# Autodesk Inventor assembly: Mass 2, 3 Group
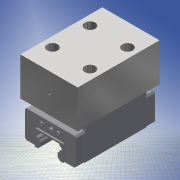
[picture p0: Inventor's stored thumbnail of the model, 180x180]
Saved by Autodesk Inventor 2016 (Build 200138000, 138)
## iProperties
Created: 2015-07-07
Part Number: Mass 2, 3 Group
Document SubType Name: Assembly
Designer: Dennis
Mass: 4113.68 g
Surface Area: 687.354 cm^2
Volume: 527.98 cm^3
Density: 7.79135 g/cm^3
Author: Dennis
## Documents named in this file (4)
- C:\Users\Jason\Dropbox\NI Work\NI Ball Bearing Slider Crank\CAD\Assemblies\Mass 2, 3 Group.iam
- C:\Users\Jason\Dropbox\NI Work\NI Ball Bearing Slider Crank\CAD\Mass 2, 3.ipt
- C:\Users\Jason\Dropbox\NI Work\NI Ball Bearing Slider Crank\CAD\McMaster Parts\Ball Bearing Carriage - Ball-Bearing Carriage, Threaded-Hole, for 34 mm Rail Width - 6709K21.ipt
- C:\Users\Jason\Dropbox\NI Work\NI Ball Bearing Slider Crank\CAD\McMaster Parts\M8x1.25x50.ipt
## Components (6 placed, 3 different names)
1. Mass 2, 3:1 — Mate:1, Mate:2, Mate:3, Mate:4, Mate:5, Mate:6, Mate:7, Mate:8, Mate:9, Mate:10, Mate:11
2. Ball Bearing Carriage - Ball-Bearing Carriage, Threaded-Hole, for 34 mm Rail Width - 6709K21:1 — Mate:1, Mate:2, Mate:3
3. M8x1.25x50:1 — Mate:4, Mate:8
4. M8x1.25x50:2 — Mate:5, Mate:9
5. M8x1.25x50:3 — Mate:6, Mate:10
6. M8x1.25x50:4 — Mate:7, Mate:11
## Relationships (11: Mate 11)
- Mate:1: Mass 2, 3:1 ↔ Ball Bearing Carriage - Ball-Bearing Carriage, Threaded-Hole, for 34 mm Rail Width - 6709K21:1
- Mate:2: Mass 2, 3:1 ↔ Ball Bearing Carriage - Ball-Bearing Carriage, Threaded-Hole, for 34 mm Rail Width - 6709K21:1
- Mate:3: Mass 2, 3:1 ↔ Ball Bearing Carriage - Ball-Bearing Carriage, Threaded-Hole, for 34 mm Rail Width - 6709K21:1
- Mate:4: Mass 2, 3:1 ↔ M8x1.25x50:1
- Mate:5: Mass 2, 3:1 ↔ M8x1.25x50:2
- Mate:6: Mass 2, 3:1 ↔ M8x1.25x50:3
- Mate:7: Mass 2, 3:1 ↔ M8x1.25x50:4
- Mate:8: Mass 2, 3:1 ↔ M8x1.25x50:1
- Mate:9: Mass 2, 3:1 ↔ M8x1.25x50:2
- Mate:10: Mass 2, 3:1 ↔ M8x1.25x50:3
- Mate:11: Mass 2, 3:1 ↔ M8x1.25x50:4
